# Autodesk Inventor assembly: ClampedPrintHeadAssembly
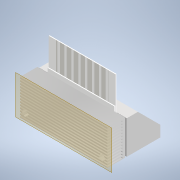
[picture p0: Inventor's stored thumbnail of the model, 180x180]
Saved by Autodesk Inventor 2021 (Build 250183000, 183)
## iProperties
Created: 2021-10-26
Part Number: ClampedPrintHeadAssembly
Document SubType Name: Assembly
Designer: Unit-005
Author: Unit-005
## Documents named in this file (6)
- C:\Users\Unit-005\Documents\Inventor\SiC_Monofilament_MicroheaterPrinthead\ClampedPrintHeadAssembly.iam
- C:\Users\Unit-005\Documents\Inventor\SiC_Monofilament_MicroheaterPrinthead\SiCMonoFilamentMicroheaterPrintHead_LessHeatSinks.iam
- C:\Users\Unit-005\Documents\Inventor\SiC_Monofilament_MicroheaterPrinthead\3DPrintedPrintHeadRetainingFrame.ipt
- C:\Users\Unit-005\Documents\Inventor\SiC_Monofilament_MicroheaterPrinthead\PreloadSPring.ipt
- C:\Users\Unit-005\Documents\Inventor\SiC_Monofilament_MicroheaterPrinthead\PrintHeadLoadPlate.ipt
- C:\Users\Unit-005\Documents\Inventor\SiC_Monofilament_MicroheaterPrinthead\ExternalHeatSinkandClamp.ipt
## Components (15 placed, 5 different names)
1. SiCMonoFilamentMicroheaterPrintHead_LessHeatSinks:1 [sub-assembly] — Flush:4, Mate:4, Flush:7, Mate:7
2. 3DPrintedPrintHeadRetainingFrame:2 — Mate:1, Flush:4, Mate:3, Flush:5, Flush:6, Mate:5, Mate:8, Flush:8
3. PrintHeadLoadPlate:2 — Mate:4, Flush:5, Mate:5
4. ExternalHeatSinkandClamp:1 — Mate:7, Mate:8, Flush:8
5. PreloadSPring:1 — Mate:3, Flush:6, Flush:7, Mate:6
6. PreloadSPring:2
7. PreloadSPring:3
8. PreloadSPring:4
9. PreloadSPring:5
10. PreloadSPring:6
11. PreloadSPring:7
12. PreloadSPring:8
13. PreloadSPring:9
14. PreloadSPring:10
15. PreloadSPring:11
## Component patterns: (11 elements, first: PreloadSPring:1)
## Relationships (12: Mate 7, Flush 5)
- Mate:1: 3DPrintedPrintHeadRetainingFrame:2
- Flush:4: SiCMonoFilamentMicroheaterPrintHead_LessHeatSinks:1 ↔ 3DPrintedPrintHeadRetainingFrame:2
- Mate:3: 3DPrintedPrintHeadRetainingFrame:2 ↔ PreloadSPring:1
- Mate:4: SiCMonoFilamentMicroheaterPrintHead_LessHeatSinks:1 ↔ PrintHeadLoadPlate:2
- Flush:5: 3DPrintedPrintHeadRetainingFrame:2 ↔ PrintHeadLoadPlate:2
- Flush:6: 3DPrintedPrintHeadRetainingFrame:2 ↔ PreloadSPring:1
- Mate:5: 3DPrintedPrintHeadRetainingFrame:2 ↔ PrintHeadLoadPlate:2
- Flush:7 (2.159 mm): SiCMonoFilamentMicroheaterPrintHead_LessHeatSinks:1 ↔ PreloadSPring:1
- Mate:6: PreloadSPring:1
- Mate:7: SiCMonoFilamentMicroheaterPrintHead_LessHeatSinks:1 ↔ ExternalHeatSinkandClamp:1
- Mate:8: 3DPrintedPrintHeadRetainingFrame:2 ↔ ExternalHeatSinkandClamp:1
- Flush:8: 3DPrintedPrintHeadRetainingFrame:2 ↔ ExternalHeatSinkandClamp:1
